# Autodesk Inventor assembly: BearingUnit
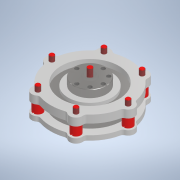
[picture p0: Inventor's stored thumbnail of the model, 180x180]
Saved by Autodesk Inventor 2020.4 (Build 244396000, 396)
## iProperties
Created: 2021-12-30
Part Number: BearingUnit
Document SubType Name: Assembly
Designer: Masato Kubotera
Mass: 95.4299 g
Surface Area: 234.903 cm^2
Volume: 20.607 cm^3
Density: 4.63094 g/cm^3
Author: Masato Kubotera
## Documents named in this file (13)
- C:\Users\Masato\Documents\Inventor\CIT Brains_Inventor\OpenPlatform_ver3_0\UpperBody\Trunk\CrossRollerBearing\BearingUnit.iam
- C:\Users\Masato\Documents\Inventor\CIT Brains_Inventor\OpenPlatform_ver3_0\ReadyMade\KONDO\ClampHorn.ipt
- C:\Users\Masato\Documents\Inventor\CIT Brains_Inventor\OpenPlatform_ver3_0\UpperBody\Trunk\CrossRollerBearing\Inner_flange.ipt
- C:\Users\Masato\Documents\Inventor\CIT Brains_Inventor\OpenPlatform_ver3_0\UpperBody\Trunk\CrossRollerBearing\Inner_support_stand.ipt
- C:\Users\Masato\Documents\Inventor\CIT Brains_Inventor\OpenPlatform_ver3_0\UpperBody\Trunk\CrossRollerBearing\Outer_flange.ipt
- C:\Users\Masato\Documents\Inventor\CIT Brains_Inventor\OpenPlatform_ver3_0\UpperBody\Trunk\CrossRollerBearing\Outer_support_stand.ipt
- C:\Users\Masato\Documents\Inventor\CIT Brains_Inventor\OpenPlatform_ver3_0\ReadyMade\Spacer\BRU-2609.5S.ipt
- C:\Users\Masato\Documents\Inventor\CIT Brains_Inventor\OpenPlatform_ver3_0\ReadyMade\InsertNut\S3-07-3W.ipt
- C:\Users\Masato\Documents\Inventor\CIT Brains_Inventor\OpenPlatform_ver3_0\ReadyMade\Screw\M2_6-6.ipt
- C:\Users\Masato\Documents\Inventor\CIT Brains_Inventor\OpenPlatform_ver3_0\ReadyMade\Screw\620103008.ipt
- C:\Users\Masato\Documents\Inventor\CIT Brains_Inventor\OpenPlatform_ver3_0\ReadyMade\Bearing\CRBA02508WWC8P5.ipt
- C:\Users\Masato\Documents\Inventor\CIT Brains_Inventor\OpenPlatform_ver3_0\ReadyMade\Spacer\BRU-309S.ipt
- C:\Users\Masato\Documents\Inventor\CIT Brains_Inventor\OpenPlatform_ver3_0\ReadyMade\Screw\M3-6.ipt
## Components (31 placed, 12 different names)
1. ClampHorn:1 — 挿入:1, 挿入:2, 挿入:3, 挿入:4, 挿入:5, 挿入:22, 角度:9, メイト:1, フラッシュ:3, メイト:2
2. Inner_flange:1 — 挿入:1, 挿入:2, 挿入:3, 挿入:4, 挿入:5, 挿入:6, 挿入:7, 挿入:8, 挿入:9, 角度:1, 角度:2, 角度:3, 角度:4, 挿入:23
3. Inner_support_stand:1 — 挿入:10, 挿入:11, 挿入:12, 挿入:13, 角度:5, 角度:6, 角度:7, 角度:8, 挿入:14, 挿入:15, 挿入:16, 挿入:17, 挿入:18, 挿入:19, 挿入:20, 挿入:21
4. BRU-2609.5S:1 — 挿入:6, 角度:1, 挿入:14
5. BRU-2609.5S:2 — 挿入:7, 角度:2, 挿入:15
6. BRU-2609.5S:3 — 挿入:8, 角度:3, 挿入:16
7. BRU-2609.5S:4 — 挿入:9, 角度:4, 挿入:17
8. S3-07-3W:1 — 挿入:10, 角度:5
9. S3-07-3W:2 — 挿入:11, 角度:6
10. S3-07-3W:3 — 挿入:12, 角度:8
11. S3-07-3W:4 — 挿入:13, 角度:7
12. CRBA02508WWC8P5:1 — 挿入:23, 挿入:24
13. Outer_flange:1 — 挿入:31, 挿入:32, 挿入:33, 挿入:34, 挿入:35, 挿入:36, 挿入:37, 挿入:38, 挿入:39, 挿入:40, 挿入:41, 挿入:42
14. Outer_support_stand:1 — 挿入:24, 角度:9, 挿入:25, 挿入:26, 挿入:27, 挿入:28, 挿入:29, 挿入:30, 角度:10, 角度:11, 角度:12, 角度:13, 角度:14, 角度:15
15. BRU-309S:1 — 挿入:25, 角度:10, 挿入:31
16. BRU-309S:2 — 挿入:26, 角度:11, 挿入:32
17. BRU-309S:3 — 挿入:27, 角度:12, 挿入:33
18. BRU-309S:4 — 挿入:28, 角度:13, 挿入:34
19. BRU-309S:5 — 挿入:29, 角度:14, 挿入:35
20. BRU-309S:6 — 挿入:30, 角度:15, 挿入:36
21. 620103008:1 — 挿入:22
22. M3-6:1 — 挿入:37
23. M3-6:2 — 挿入:38
24. M3-6:3 — 挿入:39
25. M3-6:4 — 挿入:40
26. M3-6:5 — 挿入:41
27. M3-6:6 — 挿入:42
28. M2_6-6:1 — 挿入:18
29. M2_6-6:2 — 挿入:19
30. M2_6-6:3 — 挿入:20
31. M2_6-6:4 — 挿入:21
## Relationships (60: Insert 42, Angle 15, Mate 2, Flush 1)
- 挿入:1 [Insert]: ClampHorn:1 ↔ Inner_flange:1
- 挿入:2 [Insert]: ClampHorn:1 ↔ Inner_flange:1
- 挿入:3 [Insert]: ClampHorn:1 ↔ Inner_flange:1
- 挿入:4 [Insert]: ClampHorn:1 ↔ Inner_flange:1
- 挿入:5 [Insert]: ClampHorn:1 ↔ Inner_flange:1
- 挿入:6 [Insert]: Inner_flange:1 ↔ BRU-2609.5S:1
- 挿入:7 [Insert]: Inner_flange:1 ↔ BRU-2609.5S:2
- 挿入:8 [Insert]: Inner_flange:1 ↔ BRU-2609.5S:3
- 挿入:9 [Insert]: Inner_flange:1 ↔ BRU-2609.5S:4
- 角度:1 [Angle] (0 deg): Inner_flange:1 ↔ BRU-2609.5S:1
- 角度:2 [Angle] (0 deg): Inner_flange:1 ↔ BRU-2609.5S:2
- 角度:3 [Angle] (0 deg): Inner_flange:1 ↔ BRU-2609.5S:3
- 角度:4 [Angle] (0 deg): Inner_flange:1 ↔ BRU-2609.5S:4
- 挿入:10 [Insert]: Inner_support_stand:1 ↔ S3-07-3W:1
- 挿入:11 [Insert]: Inner_support_stand:1 ↔ S3-07-3W:2
- 挿入:12 [Insert]: Inner_support_stand:1 ↔ S3-07-3W:3
- 挿入:13 [Insert]: Inner_support_stand:1 ↔ S3-07-3W:4
- 角度:5 [Angle] (0 deg): Inner_support_stand:1 ↔ S3-07-3W:1
- 角度:6 [Angle] (0 deg): Inner_support_stand:1 ↔ S3-07-3W:2
- 角度:7 [Angle] (0 deg): Inner_support_stand:1 ↔ S3-07-3W:4
- 角度:8 [Angle] (0 deg): Inner_support_stand:1 ↔ S3-07-3W:3
- 挿入:14 [Insert]: Inner_support_stand:1 ↔ BRU-2609.5S:1
- 挿入:15 [Insert]: Inner_support_stand:1 ↔ BRU-2609.5S:2
- 挿入:16 [Insert]: Inner_support_stand:1 ↔ BRU-2609.5S:3
- 挿入:17 [Insert]: Inner_support_stand:1 ↔ BRU-2609.5S:4
- 挿入:18 [Insert]: Inner_support_stand:1 ↔ M2_6-6:1
- 挿入:19 [Insert]: Inner_support_stand:1 ↔ M2_6-6:2
- 挿入:20 [Insert]: Inner_support_stand:1 ↔ M2_6-6:3
- 挿入:21 [Insert]: Inner_support_stand:1 ↔ M2_6-6:4
- 挿入:22 [Insert]: ClampHorn:1 ↔ 620103008:1
- 挿入:23 [Insert]: Inner_flange:1 ↔ CRBA02508WWC8P5:1
- 挿入:24 [Insert]: CRBA02508WWC8P5:1 ↔ Outer_support_stand:1
- 角度:9 [Angle] (90 deg): ClampHorn:1 ↔ Outer_support_stand:1
- 挿入:25 [Insert]: Outer_support_stand:1 ↔ BRU-309S:1
- 挿入:26 [Insert]: Outer_support_stand:1 ↔ BRU-309S:2
- 挿入:27 [Insert]: Outer_support_stand:1 ↔ BRU-309S:3
- 挿入:28 [Insert]: Outer_support_stand:1 ↔ BRU-309S:4
- 挿入:29 [Insert]: Outer_support_stand:1 ↔ BRU-309S:5
- 挿入:30 [Insert]: Outer_support_stand:1 ↔ BRU-309S:6
- 角度:10 [Angle] (0 deg): Outer_support_stand:1 ↔ BRU-309S:1
- 角度:11 [Angle] (0 deg): Outer_support_stand:1 ↔ BRU-309S:2
- 角度:12 [Angle] (0 deg): Outer_support_stand:1 ↔ BRU-309S:3
- 角度:13 [Angle] (0 deg): Outer_support_stand:1 ↔ BRU-309S:4
- 角度:14 [Angle] (0 deg): Outer_support_stand:1 ↔ BRU-309S:5
- 角度:15 [Angle] (0 deg): Outer_support_stand:1 ↔ BRU-309S:6
- 挿入:31 [Insert]: Outer_flange:1 ↔ BRU-309S:1
- 挿入:32 [Insert]: Outer_flange:1 ↔ BRU-309S:2
- 挿入:33 [Insert]: Outer_flange:1 ↔ BRU-309S:3
- 挿入:34 [Insert]: Outer_flange:1 ↔ BRU-309S:4
- 挿入:35 [Insert]: Outer_flange:1 ↔ BRU-309S:5
- 挿入:36 [Insert]: Outer_flange:1 ↔ BRU-309S:6
- 挿入:37 [Insert]: Outer_flange:1 ↔ M3-6:1
- 挿入:38 [Insert]: Outer_flange:1 ↔ M3-6:2
- 挿入:39 [Insert]: Outer_flange:1 ↔ M3-6:3
- 挿入:40 [Insert]: Outer_flange:1 ↔ M3-6:4
- 挿入:41 [Insert]: Outer_flange:1 ↔ M3-6:5
- 挿入:42 [Insert]: Outer_flange:1 ↔ M3-6:6
- メイト:1 [Mate]: ClampHorn:1
- フラッシュ:3 [Flush]: ClampHorn:1
- メイト:2 [Mate]: ClampHorn:1
